# Autodesk Inventor assembly: Assembly1
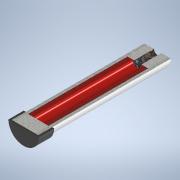
[picture p0: Inventor's stored thumbnail of the model, 180x180]
Saved by Autodesk Inventor 2021 (Build 250183000, 183)
## iProperties
Created: 2021-04-18
Part Number: Assembly1
Document SubType Name: Assembly
Designer: samlo
Author: samlo
## Documents named in this file (7)
- C:\Users\samlo\Documents\N1-motor\Drawings\Assembly1.iam
- C:\Users\samlo\Documents\N1-motor\Drawings\casing.ipt
- C:\Users\samlo\Documents\N1-motor\Drawings\nozzle.ipt
- C:\Users\samlo\Documents\N1-motor\Drawings\grain.ipt
- C:\Users\samlo\Documents\N1-motor\Drawings\insulation.ipt
- C:\Users\samlo\Documents\N1-motor\Drawings\bulkhead.ipt
- C:\Users\samlo\Documents\N1-motor\Drawings\endcap.ipt
## Components (6 placed, 6 different names)
1. casing:1 — Mate:1, Mate:2, Mate:5, Mate:7, Mate:8
2. nozzle:1 — Mate:1, Mate:2, Mate:3, Mate:4
3. grain:1 — Mate:4
4. insulation:1 — Mate:3, Mate:6
5. bulkhead:1 — Mate:5, Mate:6
6. endcap:1 — Mate:7, Mate:8
## Relationships (8: Mate 8)
- Mate:1: casing:1 ↔ nozzle:1
- Mate:2: casing:1 ↔ nozzle:1
- Mate:3: nozzle:1 ↔ insulation:1
- Mate:4: nozzle:1 ↔ grain:1
- Mate:5: casing:1 ↔ bulkhead:1
- Mate:6: insulation:1 ↔ bulkhead:1
- Mate:7: casing:1 ↔ endcap:1
- Mate:8: casing:1 ↔ endcap:1
